# Autodesk Inventor assembly: PCBsUnit
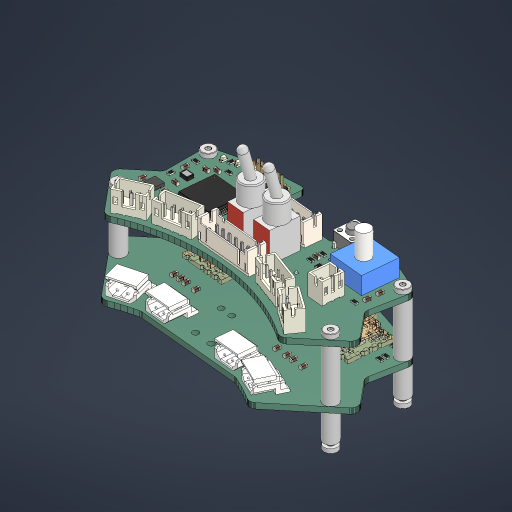
[picture p0: Inventor's stored thumbnail of the model, 512x512]
Saved by Autodesk Inventor 2024.2 (Build 282272000, 272)
## iProperties
Created: 2023-12-28
Part Number: PCBsUnit
Document SubType Name: Assembly
Designer: Hanaoka
Author: Hanaoka
## Documents named in this file (8)
- G:\共有ドライブ\reRo\05_個人\hanaoka\inventor\PCBs\PCBsUnit.iam
- G:\共有ドライブ\reRo\05_個人\hanaoka\inventor\PCBs\MotorDriver_v2\MotorDriver_v2.iam
- G:\共有ドライブ\reRo\05_個人\hanaoka\inventor\Spacer\Spacer_M2x8.ipt
- G:\共有ドライブ\reRo\05_個人\hanaoka\inventor\PCBs\MainMCU_PCB.ipt
- G:\共有ドライブ\reRo\05_個人\hanaoka\inventor\PCBs\MotorDriver_PCB.ipt
- G:\共有ドライブ\reRo\05_個人\hanaoka\inventor\Screw\M2xL6\M2x6.ipt
- G:\共有ドライブ\reRo\05_個人\hanaoka\inventor\PCBs\MainBoard_v2\MainBoard_v2.iam
- G:\共有ドライブ\reRo\05_個人\hanaoka\inventor\Spacer\Spacer_M2x15.ipt
## Components (20 placed, 7 different names)
1. MotorDriver_v2:1 [sub-assembly] — フラッシュ:1, メイト:4, 正接:2
2. Spacer_M2x8:1 — 挿入:2, 挿入:13
3. Spacer_M2x8:2 — 挿入:1, 挿入:12
4. Spacer_M2x8:3 — 挿入:4, 挿入:14
5. Spacer_M2x8:4 — 挿入:3, 挿入:11
6. MainMCU_PCB:1 — 挿入:1, 挿入:2, 挿入:3, 挿入:4, メイト:2, メイト:3, 正接:1, フラッシュ:1, メイト:4, 正接:2
7. MotorDriver_PCB:1 — 挿入:15, 挿入:16, 挿入:17, 挿入:18, フラッシュ:6, フラッシュ:7, フラッシュ:8
8. Spacer_M2x15:1
9. Spacer_M2x15:2
10. Spacer_M2x15:3
11. Spacer_M2x15:4
12. M2x6:1 — 挿入:18
13. M2x6:2 — 挿入:13
14. M2x6:3 — 挿入:11
15. M2x6:4 — 挿入:17
16. M2x6:5 — 挿入:12
17. M2x6:6 — 挿入:14
18. M2x6:7 — 挿入:16
19. M2x6:8 — 挿入:15
20. MainBoard_v2:1 [sub-assembly] — フラッシュ:6, フラッシュ:7, フラッシュ:8
## Relationships (27: Insert 18, Flush 4, Mate 3, Tangent 2)
- 挿入:1 [Insert]: Spacer_M2x8:2 ↔ MainMCU_PCB:1
- 挿入:2 [Insert]: Spacer_M2x8:1 ↔ MainMCU_PCB:1
- 挿入:3 [Insert]: Spacer_M2x8:4 ↔ MainMCU_PCB:1
- 挿入:4 [Insert]: Spacer_M2x8:3 ↔ MainMCU_PCB:1
- [Insert]: MainMCU_PCB:1 ↔ Spacer_M2x15:1
- [Insert]: MainMCU_PCB:1 ↔ Spacer_M2x15:3
- [Insert]: MainMCU_PCB:1 ↔ Spacer_M2x15:4
- [Insert]: MainMCU_PCB:1 ↔ Spacer_M2x15:2
- [Insert]: MotorDriver_PCB:1 ↔ Spacer_M2x15:2
- [Insert]: MotorDriver_PCB:1 ↔ Spacer_M2x15:1
- 挿入:11 [Insert] (1 mm): Spacer_M2x8:4 ↔ M2x6:3
- 挿入:12 [Insert] (1 mm): Spacer_M2x8:2 ↔ M2x6:5
- 挿入:13 [Insert] (1 mm): Spacer_M2x8:1 ↔ M2x6:2
- 挿入:14 [Insert] (1 mm): Spacer_M2x8:3 ↔ M2x6:6
- 挿入:15 [Insert]: MotorDriver_PCB:1 ↔ M2x6:8
- 挿入:16 [Insert]: MotorDriver_PCB:1 ↔ M2x6:7
- 挿入:17 [Insert]: MotorDriver_PCB:1 ↔ M2x6:4
- 挿入:18 [Insert]: MotorDriver_PCB:1 ↔ M2x6:1
- メイト:2 [Mate]: MainMCU_PCB:1
- メイト:3 [Mate]: MainMCU_PCB:1
- 正接:1 [Tangent]: MainMCU_PCB:1
- フラッシュ:1 [Flush]: MotorDriver_v2:1 ↔ MainMCU_PCB:1
- メイト:4 [Mate] (-1.6 mm): MotorDriver_v2:1 ↔ MainMCU_PCB:1
- 正接:2 [Tangent]: MotorDriver_v2:1 ↔ MainMCU_PCB:1
- フラッシュ:6 [Flush]: MotorDriver_PCB:1 ↔ MainBoard_v2:1
- フラッシュ:7 [Flush]: MotorDriver_PCB:1 ↔ MainBoard_v2:1
- フラッシュ:8 [Flush]: MotorDriver_PCB:1 ↔ MainBoard_v2:1
